# Autodesk Inventor assembly: 回路ボックス
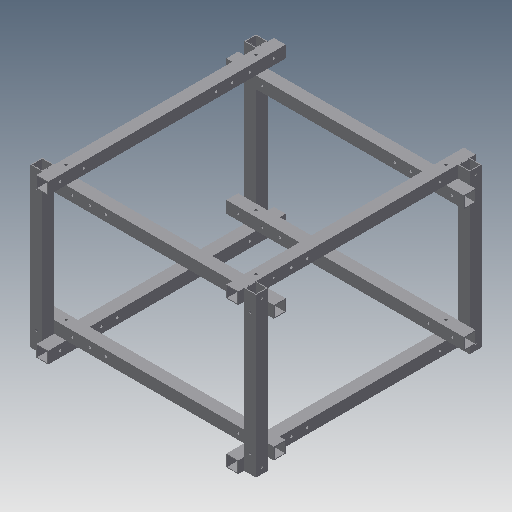
[picture p0: Inventor's stored thumbnail of the model, 512x512]
Saved by Autodesk Inventor 2019.4 (Build 234330000, 330)
## iProperties
Created: 2018-06-23
Part Number: 回路ボックス
Material: 一般
Document SubType Name: Assembly
Designer: AzLIer
Mass: 178.428 g
Surface Area: 3591.65 cm^2
Volume: 178.428 cm^3
Density: 1 g/cm^3
Author: AzLIer
## Documents named in this file (3)
- E:\ロボ研\キャチロボ\キャチロボ2018\アーム\アーム01\回路ボックス.iam
- E:\ロボ研\キャチロボ\キャチロボ2018\アーム\アーム01\回路角柱.ipt
- E:\ロボ研\キャチロボ\キャチロボ2018\アーム\アーム01\回路角柱L200.ipt
## Components (12 placed, 2 different names)
1. 回路角柱:1 — メイト:1, フラッシュ:1, 挿入:1, 挿入:4
2. 回路角柱:2 — メイト:1, フラッシュ:1, 挿入:2, 挿入:3, 挿入:5, 挿入:7
3. 回路角柱:3 — 挿入:3, 挿入:4, 挿入:6
4. 回路角柱:4 — 挿入:1, 挿入:2, 挿入:8
5. 回路角柱L200:1 — 挿入:5, 挿入:6, 挿入:13, 挿入:23
6. 回路角柱L200:2 — 挿入:7, 挿入:8, 挿入:14
7. 回路角柱:5 — 挿入:13, 挿入:14, 挿入:17
8. 回路角柱:6 — 挿入:18, リジッド:3
9. 回路角柱:7 — リジッド:2, リジッド:3
10. 回路角柱:8 — 挿入:17, 挿入:18, 挿入:23, リジッド:1
11. 回路角柱L200:4 — リジッド:1
12. 回路角柱L200:5 — リジッド:2
## Relationships (18: Insert 13, WeldJoint 3, Mate 1, Flush 1)
- メイト:1 [Mate] (225 mm): 回路角柱:1 ↔ 回路角柱:2
- フラッシュ:1 [Flush]: 回路角柱:1 ↔ 回路角柱:2
- 挿入:1 [Insert]: 回路角柱:1 ↔ 回路角柱:4
- 挿入:2 [Insert]: 回路角柱:2 ↔ 回路角柱:4
- 挿入:3 [Insert]: 回路角柱:2 ↔ 回路角柱:3
- 挿入:4 [Insert]: 回路角柱:1 ↔ 回路角柱:3
- 挿入:5 [Insert]: 回路角柱:2 ↔ 回路角柱L200:1
- 挿入:6 [Insert]: 回路角柱:3 ↔ 回路角柱L200:1
- 挿入:7 [Insert]: 回路角柱:2 ↔ 回路角柱L200:2
- 挿入:8 [Insert]: 回路角柱:4 ↔ 回路角柱L200:2
- 挿入:13 [Insert]: 回路角柱L200:1 ↔ 回路角柱:5
- 挿入:14 [Insert]: 回路角柱L200:2 ↔ 回路角柱:5
- 挿入:17 [Insert]: 回路角柱:5 ↔ 回路角柱:8
- 挿入:18 [Insert]: 回路角柱:6 ↔ 回路角柱:8
- 挿入:23 [Insert]: 回路角柱L200:1 ↔ 回路角柱:8
- リジッド:1 [WeldJoint]: 回路角柱:8 ↔ 回路角柱L200:4
- リジッド:2 [WeldJoint]: 回路角柱:7 ↔ 回路角柱L200:5
- リジッド:3 [WeldJoint]: 回路角柱:6 ↔ 回路角柱:7
